# Autodesk Inventor assembly: ensamble2
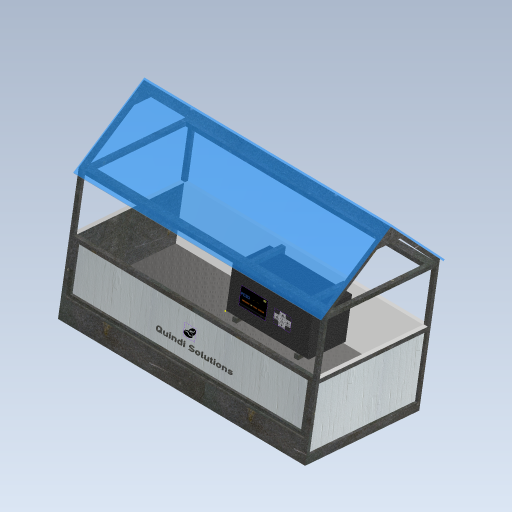
[picture p0: Inventor's stored thumbnail of the model, 512x512]
Saved by Autodesk Inventor 2023 (Build 270158000, 158)
## iProperties
Created: 2023-03-08
Part Number: ensamble2
Document SubType Name: Assembly
Designer: santi
Author: santi
## Documents named in this file (9)
- D:\u_quindio\6. Sexto semestre\cdio3\diseño2\ensamble2\ensamble2.iam
- D:\u_quindio\6. Sexto semestre\cdio3\diseño2\estructuragen\estructuragen.ipt
- D:\u_quindio\6. Sexto semestre\cdio3\diseño2\caja\caja.ipt
- D:\u_quindio\6. Sexto semestre\cdio3\diseño2\techo\techo.ipt
- D:\u_quindio\6. Sexto semestre\cdio3\diseño2\celda\celda.ipt
- D:\u_quindio\6. Sexto semestre\cdio3\diseño2\placa\placa.ipt
- D:\u_quindio\6. Sexto semestre\cdio3\diseño2\puerta\puerta.ipt
- D:\u_quindio\6. Sexto semestre\cdio3\diseño2\alza\alza.ipt
- D:\u_quindio\6. Sexto semestre\cdio3\diseño2\resorte\resorte.ipt
## Components (11 placed, 8 different names)
1. estructuragen:1 — Mate:2, Mate:3, Mate:4, Mate:5, Mate:6, Mate:7, Mate:18, Mate:19, Mate:21, Mate:22, Angle:1, Mate:23, Mate:24, Mate:29, Mate:31, Mate:32, Mate:33, Mate:34
2. caja:2 — Mate:5, Mate:6, Mate:7
3. techo:1 — Mate:2, Mate:3, Mate:4
4. celda:1 — Mate:23, Mate:24, Mate:26, Mate:27, Mate:28, Mate:29
5. placa:1 — Mate:18, Mate:19, Mate:30
6. puerta:1 — Mate:21, Mate:22, Angle:1
7. alza:1 — Mate:26, Mate:27, Mate:28, Mate:30
8. resorte:1 — Mate:31
9. resorte:2 — Mate:33
10. resorte:3 — Mate:32
11. resorte:4 — Mate:34
## Relationships (22: Mate 21, Angle 1)
- Mate:2: estructuragen:1 ↔ techo:1
- Mate:3: estructuragen:1 ↔ techo:1
- Mate:4: estructuragen:1 ↔ techo:1
- Mate:5: estructuragen:1 ↔ caja:2
- Mate:6: estructuragen:1 ↔ caja:2
- Mate:7 (10 mm): estructuragen:1 ↔ caja:2
- Mate:18: estructuragen:1 ↔ placa:1
- Mate:19: estructuragen:1 ↔ placa:1
- Mate:21: estructuragen:1 ↔ puerta:1
- Mate:22: estructuragen:1 ↔ puerta:1
- Angle:1 (0 deg): estructuragen:1 ↔ puerta:1
- Mate:23: estructuragen:1 ↔ celda:1
- Mate:24: estructuragen:1 ↔ celda:1
- Mate:26: celda:1 ↔ alza:1
- Mate:27: celda:1 ↔ alza:1
- Mate:28: celda:1 ↔ alza:1
- Mate:29: estructuragen:1 ↔ celda:1
- Mate:30: placa:1 ↔ alza:1
- Mate:31: estructuragen:1 ↔ resorte:1
- Mate:32: estructuragen:1 ↔ resorte:3
- Mate:33: estructuragen:1 ↔ resorte:2
- Mate:34: estructuragen:1 ↔ resorte:4
